# Autodesk Inventor assembly: ASY MSC 202 LEFT BOARD
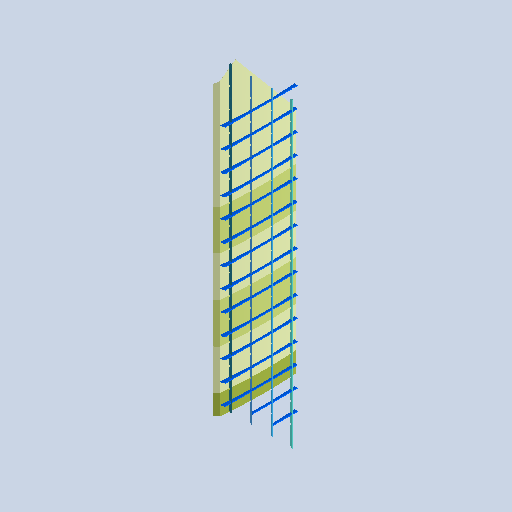
[picture p0: Inventor's stored thumbnail of the model, 512x512]
Saved by Autodesk Inventor 2025 (Build 290162010, 162A)
## iProperties
Created: 2024-07-21
Part Number: ASY MSC 202 LEFT BOARD
Document SubType Name: Assembly
Designer: pokla
Author: pokla
## Documents named in this file (13)
- C:\Users\pokla\Documents\Inventor\Отстойник осветлитель\Manturovo_Se-clar-Gleb\ASY MSC 202 LEFT BOARD.iam
- C:\Users\pokla\Documents\Inventor\Отстойник осветлитель\Manturovo_Se-clar-Gleb\MSC 052 rib board.ipt
- C:\Users\pokla\Documents\Inventor\Отстойник осветлитель\Manturovo_Se-clar-Gleb\MSC 024 sheet board main.ipt
- C:\Users\pokla\Documents\Inventor\Отстойник осветлитель\Manturovo_Se-clar-Gleb\MSC 023 sheet board.ipt
- C:\Users\pokla\Documents\Inventor\Отстойник осветлитель\Manturovo_Se-clar-Gleb\MSC 063 stringer board #.ipt
- C:\Users\pokla\Documents\Inventor\Отстойник осветлитель\Manturovo_Se-clar-Gleb\MSC 064 stringer board ##.ipt
- C:\Users\pokla\Documents\Inventor\Отстойник осветлитель\Manturovo_Se-clar-Gleb\MSC 065 stringer board ###.ipt
- C:\Users\pokla\Documents\Inventor\Отстойник осветлитель\Manturovo_Se-clar-Gleb\MSC 066 stringer board ####.ipt
- C:\Users\pokla\Documents\Inventor\Отстойник осветлитель\Manturovo_Se-clar-Gleb\MSC 025 sheet board withers 1.ipt
- C:\Users\pokla\Documents\Inventor\Отстойник осветлитель\Manturovo_Se-clar-Gleb\MSC 027 sheet board face 1.ipt
- C:\Users\pokla\Documents\Inventor\Отстойник осветлитель\Manturovo_Se-clar-Gleb\MSC 055 rib hip 2.ipt
- C:\Users\pokla\Documents\Inventor\Отстойник осветлитель\Manturovo_Se-clar-Gleb\MSC 054 rib hip 1.ipt
- C:\Users\pokla\Documents\Inventor\Отстойник осветлитель\Manturovo_Se-clar-Gleb\MSC 0512 rib back mould left board.ipt
## Components (55 placed, 17 different names)
1. MSC 052 rib board.ipt:3 — Rigid:16, Rigid:17, Flush:1, Flush:2, Flush:3
2. MSC 024 sheet board main.ipt:1 — Rigid:19, Flush:7
3. MSC 024 sheet board main.ipt:2
4. MSC 024 sheet board main.ipt:3
5. MSC 024 sheet board main.ipt:4
6. MSC 024 sheet board main.ipt:5
7. MSC 023 sheet board.ipt:1 — Flush:1, Flush:2, Flush:3, Rigid:19
8. MSC 063 stringer board #.ipt:2
9. MSC 064 stringer board ##.ipt:2
10. MSC 065 stringer board ###.ipt:2
11. MSC 066 stringer board ####.ipt:2
12. MSC 025 sheet board withers 1.ipt:1
13. MSC 027 sheet board face 1.ipt:1
14. MSC 052 rib board.ipt:5 — Rigid:16, Rigid:20
15. MSC 063 stringer board #.ipt:3 — Rigid:41
16. MSC 064 stringer board ##.ipt:3 — Rigid:38
17. MSC 065 stringer board ###.ipt:3 — Rigid:35
18. MSC 066 stringer board ####.ipt:3 — Rigid:32
19. MSC 055 rib hip 2:1 — Rigid:17, Rigid:18
20. MSC 054 rib board hip 1:1 — Rigid:18
21. MSC 0512 rib back mould left board:1 — Flush:4, Flush:6, Flush:7, Rigid:44, Rigid:55
22. MSC 052 rib board:4 — Rigid:20, Rigid:21
23. MSC 052 rib board:6 — Rigid:21, Rigid:22
24. MSC 052 rib board:7 — Rigid:22, Rigid:25
25. MSC 052 rib board:8 — Rigid:25
26. MSC 052 rib board:9
27. MSC 052 rib board:10 — Rigid:31
28. MSC 052 rib board:11 — Rigid:31
29. MSC 052 rib board:12
30. MSC 052 rib board:13
31. MSC 052 rib board:14
32. MSC 052 rib board:15
33. МОО 056 стрингер борт 6:4 — Rigid:32, Rigid:33
34. МОО 056 стрингер борт 6:5 — Rigid:33, Rigid:34
35. МОО 056 стрингер борт 6:6 — Rigid:34
36. МОО 055 стрингер борт 5:4 — Rigid:35, Rigid:36
37. МОО 055 стрингер борт 5:5 — Rigid:36, Rigid:37
38. МОО 055 стрингер борт 5:6 — Rigid:37
39. МОО 054 стрингер борт 4:4 — Rigid:38, Rigid:39
40. МОО 054 стрингер борт 4:5 — Rigid:39, Rigid:40
41. МОО 054 стрингер борт 4:6 — Rigid:40
42. МОО 053 стрингер борт 3:4 — Rigid:41, Rigid:42
43. МОО 053 стрингер борт 3:5 — Rigid:42, Rigid:43
44. МОО 053 стрингер борт 3:6 — Rigid:43
45. MSC 0512 rib back mould left board:2 — Rigid:44, Rigid:45
46. MSC 0512 rib back mould left board:3 — Rigid:45, Rigid:47
47. MSC 0512 rib back mould left board:4 — Rigid:47
48. MSC 0512 rib back mould left board:5 — Rigid:51
49. MSC 0512 rib back mould left board:6 — Rigid:51
50. MSC 0512 rib back mould left board:7
51. MSC 0512 rib back mould left board:8
52. MSC 0512 rib back mould left board:9 — Rigid:54
53. MSC 0512 rib back mould left board:10 — Rigid:54
54. MSC 0512 rib back mould left board:11
55. MSC 0512 rib back mould left board:12 — Rigid:55
## Relationships (59: WeldJoint 52, Flush 6, Mate 1)
- [WeldJoint]: MSC 024 sheet board main.ipt:1 ↔ MSC 024 sheet board main.ipt:2
- [WeldJoint]: MSC 024 sheet board main.ipt:2 ↔ MSC 024 sheet board main.ipt:3
- [WeldJoint]: MSC 024 sheet board main.ipt:3 ↔ MSC 024 sheet board main.ipt:4
- [WeldJoint]: MSC 024 sheet board main.ipt:4 ↔ MSC 024 sheet board main.ipt:5
- [Mate]: MSC 024 sheet board main.ipt:1 ↔ MSC 023 sheet board.ipt:1
- [WeldJoint]: MSC 024 sheet board main.ipt:5 ↔ MSC 025 sheet board withers 1.ipt:1
- [WeldJoint]: MSC 025 sheet board withers 1.ipt:1 ↔ MSC 027 sheet board face 1.ipt:1
- [WeldJoint] (2 mm): MSC 052 rib board.ipt:3 ↔ MSC 066 stringer board ####.ipt:2
- [WeldJoint]: MSC 063 stringer board #.ipt:2 ↔ MSC 063 stringer board #.ipt:3
- [WeldJoint]: MSC 064 stringer board ##.ipt:2 ↔ MSC 064 stringer board ##.ipt:3
- [WeldJoint]: MSC 065 stringer board ###.ipt:2 ↔ MSC 065 stringer board ###.ipt:3
- [WeldJoint]: MSC 066 stringer board ####.ipt:2 ↔ MSC 066 stringer board ####.ipt:3
- [WeldJoint] (2 mm): MSC 052 rib board.ipt:3 ↔ MSC 065 stringer board ###.ipt:2
- [WeldJoint] (2 mm): MSC 052 rib board.ipt:3 ↔ MSC 064 stringer board ##.ipt:2
- [WeldJoint] (2 mm): MSC 052 rib board.ipt:3 ↔ MSC 063 stringer board #.ipt:3
- Rigid:16 [WeldJoint] (-500 mm): MSC 052 rib board.ipt:3 ↔ MSC 052 rib board.ipt:5
- Rigid:17 [WeldJoint] (500 mm): MSC 052 rib board.ipt:3 ↔ MSC 055 rib hip 2:1
- Rigid:18 [WeldJoint] (500 mm): MSC 055 rib hip 2:1 ↔ MSC 054 rib board hip 1:1
- Flush:1 (248 mm): MSC 052 rib board.ipt:3 ↔ MSC 023 sheet board.ipt:1
- Flush:2: MSC 052 rib board.ipt:3 ↔ MSC 023 sheet board.ipt:1
- Flush:3: MSC 052 rib board.ipt:3 ↔ MSC 023 sheet board.ipt:1
- Rigid:19 [WeldJoint]: MSC 024 sheet board main.ipt:1 ↔ MSC 023 sheet board.ipt:1
- Rigid:20 [WeldJoint] (-500 mm): MSC 052 rib board.ipt:5 ↔ MSC 052 rib board:4
- Rigid:21 [WeldJoint] (-500 mm): MSC 052 rib board:4 ↔ MSC 052 rib board:6
- Rigid:22 [WeldJoint] (-500 mm): MSC 052 rib board:6 ↔ MSC 052 rib board:7
- [WeldJoint] (-500 mm): MSC 052 rib board:8 ↔ MSC 052 rib board:9
- [WeldJoint] (-500 mm): MSC 052 rib board:9 ↔ MSC 052 rib board:10
- Rigid:25 [WeldJoint] (-500 mm): MSC 052 rib board:7 ↔ MSC 052 rib board:8
- [WeldJoint] (-500 mm): MSC 052 rib board:11 ↔ MSC 052 rib board:12
- [WeldJoint] (-500 mm): MSC 052 rib board:12 ↔ MSC 052 rib board:13
- [WeldJoint] (-500 mm): MSC 052 rib board:14 ↔ MSC 052 rib board:15
- [WeldJoint] (-500 mm): MSC 052 rib board:13 ↔ MSC 052 rib board:14
- Rigid:31 [WeldJoint] (-500 mm): MSC 052 rib board:10 ↔ MSC 052 rib board:11
- Rigid:32 [WeldJoint]: MSC 066 stringer board ####.ipt:3 ↔ МОО 056 стрингер борт 6:4
- Rigid:33 [WeldJoint]: МОО 056 стрингер борт 6:4 ↔ МОО 056 стрингер борт 6:5
- Rigid:34 [WeldJoint]: МОО 056 стрингер борт 6:5 ↔ МОО 056 стрингер борт 6:6
- Rigid:35 [WeldJoint]: MSC 065 stringer board ###.ipt:3 ↔ МОО 055 стрингер борт 5:4
- Rigid:36 [WeldJoint]: МОО 055 стрингер борт 5:4 ↔ МОО 055 стрингер борт 5:5
- Rigid:37 [WeldJoint]: МОО 055 стрингер борт 5:5 ↔ МОО 055 стрингер борт 5:6
- Rigid:38 [WeldJoint]: MSC 064 stringer board ##.ipt:3 ↔ МОО 054 стрингер борт 4:4
- Rigid:39 [WeldJoint]: МОО 054 стрингер борт 4:4 ↔ МОО 054 стрингер борт 4:5
- Rigid:40 [WeldJoint]: МОО 054 стрингер борт 4:5 ↔ МОО 054 стрингер борт 4:6
- Rigid:41 [WeldJoint]: MSC 063 stringer board #.ipt:3 ↔ МОО 053 стрингер борт 3:4
- Rigid:42 [WeldJoint]: МОО 053 стрингер борт 3:4 ↔ МОО 053 стрингер борт 3:5
- Rigid:43 [WeldJoint]: МОО 053 стрингер борт 3:5 ↔ МОО 053 стрингер борт 3:6
- Flush:4: MSC 0512 rib back mould left board:1
- Flush:6: MSC 0512 rib back mould left board:1
- Flush:7 (248.5 mm): MSC 024 sheet board main.ipt:1 ↔ MSC 0512 rib back mould left board:1
- Rigid:44 [WeldJoint] (497 mm): MSC 0512 rib back mould left board:1 ↔ MSC 0512 rib back mould left board:2
- Rigid:45 [WeldJoint] (497 mm): MSC 0512 rib back mould left board:2 ↔ MSC 0512 rib back mould left board:3
- [WeldJoint] (497 mm): MSC 0512 rib back mould left board:4 ↔ MSC 0512 rib back mould left board:5
- Rigid:47 [WeldJoint] (497 mm): MSC 0512 rib back mould left board:3 ↔ MSC 0512 rib back mould left board:4
- [WeldJoint] (497 mm): MSC 0512 rib back mould left board:6 ↔ MSC 0512 rib back mould left board:7
- [WeldJoint] (497 mm): MSC 0512 rib back mould left board:8 ↔ MSC 0512 rib back mould left board:9
- [WeldJoint] (497 mm): MSC 0512 rib back mould left board:7 ↔ MSC 0512 rib back mould left board:8
- Rigid:51 [WeldJoint] (497 mm): MSC 0512 rib back mould left board:5 ↔ MSC 0512 rib back mould left board:6
- [WeldJoint] (497 mm): MSC 0512 rib back mould left board:10 ↔ MSC 0512 rib back mould left board:11
- Rigid:54 [WeldJoint] (497 mm): MSC 0512 rib back mould left board:9 ↔ MSC 0512 rib back mould left board:10
- Rigid:55 [WeldJoint] (497 mm): MSC 0512 rib back mould left board:1 ↔ MSC 0512 rib back mould left board:12
## Named parameters: d29_d27 = -500 mm, d30_d28 = -500 mm, d32_d27 = -500 mm, d33_d28 = -500 mm, d34_d29_d27 = -500 mm, d36_d31 = -500 mm, d56_d55 = 497 mm, d58_d55 = 497 mm, d59_d56_d55 = 497 mm, d60_d57 = 497 mm, d63_d60_d57 = 497 mm
